# Autodesk Inventor assembly: ZlozenieDwochSuperCzesci
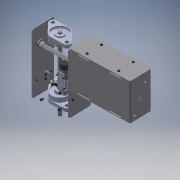
[picture p0: Inventor's stored thumbnail of the model, 180x180]
Saved by Autodesk Inventor 2019 (Build 230136000, 136)
## iProperties
Created: 2020-08-29
Part Number: ZlozenieDwochSuperCzesci
Document SubType Name: Assembly
Designer: estee
Author: estee
## Documents named in this file (4)
- C:\Users\estee\OneDrive\Pulpit\estere\1\MUM\nowygit\Mechanika\Moduł obrotu DEK Bartek\odBartka\ZlozenieDwochSuperCzesci.iam
- C:\Users\estee\OneDrive\Pulpit\estere\1\MUM\nowygit\Mechanika\Moduł obrotu DEK Bartek\odBartka\Moduł1.iam
- C:\Users\estee\OneDrive\Pulpit\estere\1\MUM\nowygit\Mechanika\Moduł obrotu DEK Bartek\odBartka\Moduł3.iam
- C:\Users\estee\OneDrive\Dokumenty\Inventor\Content Center Files\R2019\en-US\ISO 4026\ISO 4026 - M3 x 3 - ISO.ipt
## Components (6 placed, 3 different names)
1. Moduł1:1 [sub-assembly] — Mate:1, Angle:1, Flush:1, Tangent:1, Tangent:2, Tangent:3, Tangent:4
2. Moduł3:1 [sub-assembly] — Mate:1, Angle:1, Flush:1, Mate:2, Mate:3, Mate:4, Mate:5
3. ISO 4026 M3 x 3:1 — Mate:5, Tangent:4
4. ISO 4026 M3 x 3:2 — Mate:2, Tangent:1
5. ISO 4026 M3 x 3:3 — Mate:3, Tangent:2
6. ISO 4026 M3 x 3:4 — Mate:4, Tangent:3
## Relationships (11: Mate 5, Tangent 4, Angle 1, Flush 1)
- Mate:1: Moduł1:1 ↔ Moduł3:1
- Angle:1 (0 deg): Moduł1:1 ↔ Moduł3:1
- Flush:1: Moduł1:1 ↔ Moduł3:1
- Mate:2: Moduł3:1 ↔ ISO 4026 M3 x 3:2
- Tangent:1: Moduł1:1 ↔ ISO 4026 M3 x 3:2
- Mate:3: Moduł3:1 ↔ ISO 4026 M3 x 3:3
- Tangent:2: Moduł1:1 ↔ ISO 4026 M3 x 3:3
- Mate:4: Moduł3:1 ↔ ISO 4026 M3 x 3:4
- Mate:5: Moduł3:1 ↔ ISO 4026 M3 x 3:1
- Tangent:3: Moduł1:1 ↔ ISO 4026 M3 x 3:4
- Tangent:4: Moduł1:1 ↔ ISO 4026 M3 x 3:1
